# Autodesk Inventor assembly: ToolHeadAssy
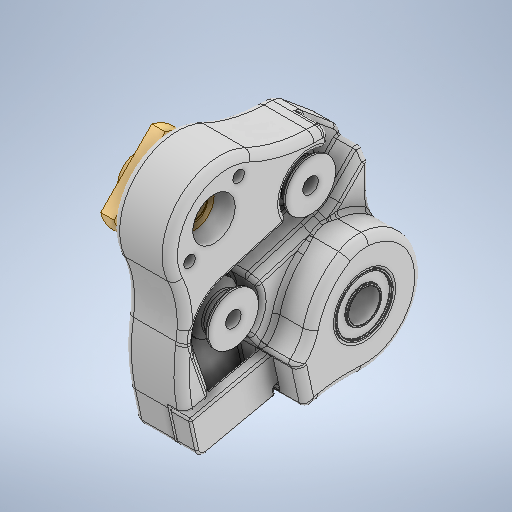
[picture p0: Inventor's stored thumbnail of the model, 512x512]
Saved by Autodesk Inventor 2025.3 (Build 293356030, 356C)
## iProperties
Created: 2025-10-22
Part Number: ToolHeadAssy
Document SubType Name: Assembly
Designer: tvoko
Author: tvoko
## iProperties of the stored document 3.Linear Bearing-LM8UU.ipt
Created: 2022-04-19
Part Number: 3.Linear Bearing-LM8UU
Material: Generic
Description: STEP AP203
Document SubType Name: Modeling
Designer: tvoko
Density: 1 g/cm^3
Appearance: Default
Sending System: SolidWorks 2017
Preprocessor: SwSTEP 2.0
Title: 3.Linear Bearing-LM8UU.STEP
Revision Number: ANY
## Documents named in this file (7)
- C:\Users\tvoko\Github\DIY-Coil-Winder\CAD\ToolHeadAssy.iam
- C:\Users\tvoko\Github\DIY-Coil-Winder\CAD\Imports\NEMA 17 Stepper Motor 39mm-NEMA 17 Stepper Motor 39mm\T8 Nut 1.5\T8 Nut 1.5.ipt
- C:\Users\tvoko\Github\DIY-Coil-Winder\CAD\GuideBlock.ipt
- C:\Users\tvoko\Github\DIY-Coil-Winder\CAD\Imports\uxcell_V624ZZ_4mmx13mmx6mm.ipt
- **C:\Users\tvoko\Github\DIY-Coil-Winder\CAD\ToolHeadAssy.iam*LocalDocs*xAaaaqkbaAaaaaaaaAaaaakp30d*3.Linear Bearing-LM8UU.ipt
- C:\Users\tvoko\Github\DIY-Coil-Winder\CAD\Tensioner-Clamp.ipt
- C:\Users\tvoko\Github\DIY-Coil-Winder\CAD\Imports\3.Linear Bearing-LM8UU.STEP
## Components (6 placed, 5 different names)
1. T8 Nut 1.5:1 — Mate:1, Mate:2, Mate:3
2. GuideBlock:1 — Mate:1, Mate:2, Mate:3, Mate:4, Flush:1, Mate:5, Mate:6, Mate:7, Mate:8, Mate:11, Flush:2
3. uxcell_V624ZZ_4mmx13mmx6mm:1 — Mate:6, Mate:7
4. uxcell_V624ZZ_4mmx13mmx6mm:2 — Mate:5, Mate:8
5. 3.Linear Bearing-LM8UU:2 — Mate:4, Flush:1
6. Tensioner-Clamp:1 — Mate:11, Flush:2
## Relationships (11: Mate 9, Flush 2)
- Mate:1: T8 Nut 1.5:1 ↔ GuideBlock:1
- Mate:2: T8 Nut 1.5:1 ↔ GuideBlock:1
- Mate:3: T8 Nut 1.5:1 ↔ GuideBlock:1
- Mate:4: GuideBlock:1 ↔ 3.Linear Bearing-LM8UU:2
- Flush:1: GuideBlock:1 ↔ 3.Linear Bearing-LM8UU:2
- Mate:5: GuideBlock:1 ↔ uxcell_V624ZZ_4mmx13mmx6mm:2
- Mate:6: GuideBlock:1 ↔ uxcell_V624ZZ_4mmx13mmx6mm:1
- Mate:7: GuideBlock:1 ↔ uxcell_V624ZZ_4mmx13mmx6mm:1
- Mate:8: GuideBlock:1 ↔ uxcell_V624ZZ_4mmx13mmx6mm:2
- Mate:11: GuideBlock:1 ↔ Tensioner-Clamp:1
- Flush:2: GuideBlock:1 ↔ Tensioner-Clamp:1
